# Autodesk Inventor assembly: YAxis_Carriage
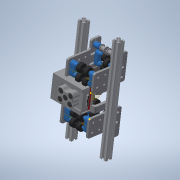
[picture p0: Inventor's stored thumbnail of the model, 180x180]
Saved by Autodesk Inventor 2021 (Build 250183000, 183)
## iProperties
Created: 2021-02-02
Part Number: YAxis_Carriage
Document SubType Name: Assembly
Designer: Jorian Brusind
Author: Jorian Brusind
## Documents named in this file (14)
- C:\Users\Jorian Brusind\Documents\GitHub\PersonalProjects\HyperRail\Inventor Files\YAxis_Carriage.iam
- C:\Users\Jorian Brusind\Documents\GitHub\PersonalProjects\Inventor Projects\Useful models\8020_Sets\IPT_20_Series\IPT_20_Series\20-2020_300mm.ipt
- C:\Users\Jorian Brusind\Documents\GitHub\PersonalProjects\Inventor Projects\Useful models\NEMA_Steppers\nema-17-stepper-motor-with-v2-damper-1.snapshot.3\Nema 17  Stepper Motor length 34mm.ipt
- C:\Users\Jorian Brusind\Documents\GitHub\PersonalProjects\Inventor Projects\Useful models\NEMA_Steppers\nema-17-steel-motor-mount-1.snapshot.2\NEMA17 - Steel Motor Mount.ipt
- C:\Users\Jorian Brusind\Documents\GitHub\PersonalProjects\HyperRail\Inventor Files\SmallBelt_Pulley.ipt
- C:\Users\Jorian Brusind\Documents\GitHub\PersonalProjects\Inventor Projects\Useful models\Metric bolt\Bolt M3 30mm.ipt
- C:\Users\Jorian Brusind\Documents\GitHub\PersonalProjects\HyperRail\Inventor Files\small_belt_loop.ipt
- C:\Users\Jorian Brusind\Documents\GitHub\PersonalProjects\HyperRail\PCB Files\Integrated Stepper Motor Driver\ExportSTEP\Main.iam
- C:\Users\Jorian Brusind\Documents\GitHub\PersonalProjects\HyperRail\Inventor Files\rededge-micasense-1.snapshot.3\PND_CAM_MSRE.ipt
- C:\Users\Jorian Brusind\Documents\GitHub\PersonalProjects\HyperRail\Inventor Files\Camera_Mount.ipt
- C:\Users\Jorian Brusind\Documents\GitHub\PersonalProjects\HyperRail\Inventor Files\X_CarriageR_V2_0.iam
- C:\Users\Jorian Brusind\Documents\GitHub\PersonalProjects\HyperRail\Inventor Files\X_Carriage_V2_0.iam
- C:\Users\Jorian Brusind\Documents\GitHub\PersonalProjects\HyperRail\Inventor Files\F623ZZ v2.iam
- C:\Users\Jorian Brusind\Documents\GitHub\PersonalProjects\HyperRail\Inventor Files\6mm_Spacer.ipt
## Components (29 placed, 13 different names)
1. 20-2020_300mm:1 — Mate:3, Flush:25, Mate:59, Flush:27, Mate:80, Mate:81, Mate:84, Flush:43
2. Nema 17  Stepper Motor length 34mm:1 — Mate:4, Mate:5, Mate:6, Mate:13, Mate:14, Mate:36, Mate:42, Flush:14, Flush:15
3. NEMA17 - Steel Motor Mount:1 — Mate:3, Mate:4, Mate:5, Mate:6, Mate:20, Mate:21, Mate:75, Mate:76, Mate:77, Mate:79, Flush:43
4. SmallBelt_Pulley:1 — Mate:13, Mate:14, Mate:37, Flush:33, Flush:34, Flush:44
5. Bolt M3 30mm:1 — Mate:20, Mate:65, Mate:66, Flush:35, Mate:94
6. Bolt M3 30mm:2 — Mate:21, Mate:38, Mate:63, Mate:64, Flush:36, Mate:95
7. small_belt_loop:1 — Mate:36, Mate:37, Mate:38
8. Main:1 [sub-assembly] — Mate:42, Flush:14, Flush:15
9. 20-2020_300mm:2 — Flush:25, Flush:26, Flush:27, Mate:82, Mate:83
10. PND_CAM_MSRE:1 — Mate:47, Mate:48, Mate:49
11. Camera_Mount:1 — Mate:47, Mate:48, Mate:49, Mate:59, Flush:26
12. F623ZZ v2:1 [sub-assembly] — Mate:65, Mate:67, Flush:34
13. F623ZZ v2:2 [sub-assembly] — Mate:66, Mate:67, Mate:99
14. F623ZZ v2:3 [sub-assembly] — Mate:63, Mate:68, Flush:33
15. F623ZZ v2:4 [sub-assembly] — Mate:64, Mate:68, Mate:96
16. Bolt M3 30mm:3 — Mate:76, Mate:78, Flush:35, Flush:36, Flush:37, Mate:88
17. F623ZZ v2:5 [sub-assembly] — Mate:78
18. F623ZZ v2:6 [sub-assembly] — Mate:77, Mate:98
19. Bolt M3 30mm:4 — Mate:75, Flush:37, Mate:93
20. F623ZZ v2:7 [sub-assembly]
21. F623ZZ v2:8 [sub-assembly] — Mate:79, Mate:97
22. X_CarriageR_V2_0:1 [sub-assembly] — Mate:82, Flush:38, Flush:39, Flush:40, Mate:85
23. X_CarriageR_V2_0:2 [sub-assembly] — Flush:40, Mate:84, Flush:42, Flush:44
24. X_Carriage_V2_0:1 [sub-assembly] — Mate:80, Mate:81, Flush:38, Flush:39, Flush:41, Mate:85
25. X_Carriage_V2_0:2 [sub-assembly] — Flush:41, Mate:83, Flush:42
26. 6mm_Spacer:1 — Mate:88, Mate:98
27. 6mm_Spacer:6 — Mate:93, Mate:97
28. 6mm_Spacer:8 — Mate:95, Mate:96
29. 6mm_Spacer:10 — Mate:94, Mate:99
## Relationships (64: Mate 47, Flush 17)
- Mate:3 (3 mm): 20-2020_300mm:1 ↔ NEMA17 - Steel Motor Mount:1
- Mate:4: Nema 17  Stepper Motor length 34mm:1 ↔ NEMA17 - Steel Motor Mount:1
- Mate:5: Nema 17  Stepper Motor length 34mm:1 ↔ NEMA17 - Steel Motor Mount:1
- Mate:6: Nema 17  Stepper Motor length 34mm:1 ↔ NEMA17 - Steel Motor Mount:1
- Mate:13: Nema 17  Stepper Motor length 34mm:1 ↔ SmallBelt_Pulley:1
- Mate:14: Nema 17  Stepper Motor length 34mm:1 ↔ SmallBelt_Pulley:1
- Mate:20: NEMA17 - Steel Motor Mount:1 ↔ Bolt M3 30mm:1
- Mate:21: NEMA17 - Steel Motor Mount:1 ↔ Bolt M3 30mm:2
- Mate:36: Nema 17  Stepper Motor length 34mm:1 ↔ small_belt_loop:1
- Mate:37 (2 mm): SmallBelt_Pulley:1 ↔ small_belt_loop:1
- Mate:38: Bolt M3 30mm:2 ↔ small_belt_loop:1
- Mate:42: Nema 17  Stepper Motor length 34mm:1 ↔ Main:1
- Flush:14: Nema 17  Stepper Motor length 34mm:1 ↔ Main:1
- Flush:15: Nema 17  Stepper Motor length 34mm:1 ↔ Main:1
- Mate:47: PND_CAM_MSRE:1 ↔ Camera_Mount:1
- Mate:48: PND_CAM_MSRE:1 ↔ Camera_Mount:1
- Mate:49: PND_CAM_MSRE:1 ↔ Camera_Mount:1
- Flush:25: 20-2020_300mm:1 ↔ 20-2020_300mm:2
- Mate:59: 20-2020_300mm:1 ↔ Camera_Mount:1
- Flush:26: 20-2020_300mm:2 ↔ Camera_Mount:1
- Flush:27: 20-2020_300mm:1 ↔ 20-2020_300mm:2
- Mate:63: Bolt M3 30mm:2 ↔ F623ZZ v2:3
- Mate:64: Bolt M3 30mm:2 ↔ F623ZZ v2:4
- Mate:65: Bolt M3 30mm:1 ↔ F623ZZ v2:1
- Mate:66: Bolt M3 30mm:1 ↔ F623ZZ v2:2
- Mate:67: F623ZZ v2:1 ↔ F623ZZ v2:2
- Mate:68: F623ZZ v2:3 ↔ F623ZZ v2:4
- Flush:33 (2 mm): SmallBelt_Pulley:1 ↔ F623ZZ v2:3
- Flush:34 (2 mm): SmallBelt_Pulley:1 ↔ F623ZZ v2:1
- [Mate]: Bolt M3 30mm:3 ↔ F623ZZ v2:5
- [Mate]: Bolt M3 30mm:3 ↔ F623ZZ v2:6
- [Mate]: F623ZZ v2:5 ↔ F623ZZ v2:6
- [Mate]: Bolt M3 30mm:4 ↔ F623ZZ v2:7
- [Mate]: Bolt M3 30mm:4 ↔ F623ZZ v2:8
- [Mate]: F623ZZ v2:7 ↔ F623ZZ v2:8
- Mate:75: NEMA17 - Steel Motor Mount:1 ↔ Bolt M3 30mm:4
- Mate:76: NEMA17 - Steel Motor Mount:1 ↔ Bolt M3 30mm:3
- Mate:77 (7 mm): NEMA17 - Steel Motor Mount:1 ↔ F623ZZ v2:6
- Mate:78: Bolt M3 30mm:3 ↔ F623ZZ v2:5
- Flush:35: Bolt M3 30mm:1 ↔ Bolt M3 30mm:3
- Flush:36: Bolt M3 30mm:2 ↔ Bolt M3 30mm:3
- Mate:79 (7 mm): NEMA17 - Steel Motor Mount:1 ↔ F623ZZ v2:8
- Flush:37: Bolt M3 30mm:3 ↔ Bolt M3 30mm:4
- Mate:80: 20-2020_300mm:1 ↔ X_Carriage_V2_0:1
- Mate:81 (5 mm): 20-2020_300mm:1 ↔ X_Carriage_V2_0:1
- Mate:82: 20-2020_300mm:2 ↔ X_CarriageR_V2_0:1
- Flush:38: X_CarriageR_V2_0:1 ↔ X_Carriage_V2_0:1
- Flush:39: X_CarriageR_V2_0:1 ↔ X_Carriage_V2_0:1
- Flush:40: X_CarriageR_V2_0:1 ↔ X_CarriageR_V2_0:2
- Flush:41: X_Carriage_V2_0:1 ↔ X_Carriage_V2_0:2
- Mate:83: 20-2020_300mm:2 ↔ X_Carriage_V2_0:2
- Mate:84: 20-2020_300mm:1 ↔ X_CarriageR_V2_0:2
- Flush:42: X_CarriageR_V2_0:2 ↔ X_Carriage_V2_0:2
- Flush:43 (120 mm): 20-2020_300mm:1 ↔ NEMA17 - Steel Motor Mount:1
- Mate:85 (10 mm): X_CarriageR_V2_0:1 ↔ X_Carriage_V2_0:1
- Flush:44: SmallBelt_Pulley:1 ↔ X_CarriageR_V2_0:2
- Mate:88: Bolt M3 30mm:3 ↔ 6mm_Spacer:1
- Mate:93: Bolt M3 30mm:4 ↔ 6mm_Spacer:6
- Mate:94: Bolt M3 30mm:1 ↔ 6mm_Spacer:10
- Mate:95: Bolt M3 30mm:2 ↔ 6mm_Spacer:8
- Mate:96: F623ZZ v2:4 ↔ 6mm_Spacer:8
- Mate:97: F623ZZ v2:8 ↔ 6mm_Spacer:6
- Mate:98: F623ZZ v2:6 ↔ 6mm_Spacer:1
- Mate:99: F623ZZ v2:2 ↔ 6mm_Spacer:10
## Named parameters: d133_d125 = 0 mm, d134_d126 = 0 mm, d135_d130 = 0 mm, d136_d125 = 0 mm, d137_d126 = 0 mm, d138_d130 = 0 mm
